# Autodesk Inventor assembly: IntakeRollerBar
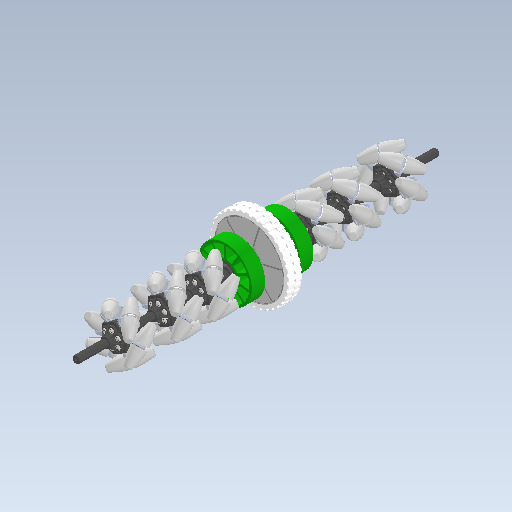
[picture p0: Inventor's stored thumbnail of the model, 512x512]
Saved by Autodesk Inventor 2020 (Build 240168000, 168)
## iProperties
Created: 2020-01-19
Part Number: IntakeRollerBar
Document SubType Name: Assembly
Designer: srini
Author: srini
## Documents named in this file (6)
- C:\Users\srini\Documents\FRC\2020\IntakeRollerBar.iam
- C:\Users\srini\Documents\FRC\2020\ThunderHex_27in.ipt
- C:\Users\srini\Documents\FRC\2020\MecWheels\4_Mecanum_Wheel_Left_217-3644.iam
- C:\Users\srini\Documents\FRC\2020\MecWheels\4_Mecanum_Wheel_Right_217-3645.iam
- C:\Users\srini\Documents\FRC\2020\am-3480 4IN 500Hex Compliant Wheel REV2.iam
- C:\Users\srini\Documents\FRC\2020\am-0940a 6 HiGrip wheel REV2_HexBore.iam
## Components (10 placed, 5 different names)
1. ThunderHex_27in:1 — Insert:1, Mate:1, Mate:3, Mate:5, Mate:7, Mate:9, Mate:11, Mate:13, Mate:15
2. 4_Mecanum_Wheel_Left_217-3644:1 [sub-assembly] — Mate:9, Mate:10
3. 4_Mecanum_Wheel_Left_217-3644:2 [sub-assembly] — Mate:7, Mate:8, Mate:10
4. 4_Mecanum_Wheel_Left_217-3644:3 [sub-assembly] — Mate:5, Mate:6, Mate:8
5. 4_Mecanum_Wheel_Right_217-3645:1 [sub-assembly] — Mate:13, Mate:14, Mate:16
6. 4_Mecanum_Wheel_Right_217-3645:2 [sub-assembly] — Mate:15, Mate:16
7. 4_Mecanum_Wheel_Right_217-3645:3 [sub-assembly] — Mate:11, Mate:12, Mate:14
8. am-3480 4IN 500Hex Compliant Wheel REV2:1 [sub-assembly] — Mate:3, Mate:4, Mate:12
9. am-3480 4IN 500Hex Compliant Wheel REV2:2 [sub-assembly] — Mate:1, Mate:2, Mate:6
10. am-0940a 6 HiGrip wheel REV2_HexBore:1 [sub-assembly] — Insert:1, Mate:2, Mate:4
## Relationships (17: Mate 16, Insert 1)
- Insert:1 (-342.9 mm): ThunderHex_27in:1 ↔ am-0940a 6 HiGrip wheel REV2_HexBore:1
- Mate:1: ThunderHex_27in:1 ↔ am-3480 4IN 500Hex Compliant Wheel REV2:2
- Mate:2 (12.7 mm): am-3480 4IN 500Hex Compliant Wheel REV2:2 ↔ am-0940a 6 HiGrip wheel REV2_HexBore:1
- Mate:3: ThunderHex_27in:1 ↔ am-3480 4IN 500Hex Compliant Wheel REV2:1
- Mate:4 (12.7 mm): am-3480 4IN 500Hex Compliant Wheel REV2:1 ↔ am-0940a 6 HiGrip wheel REV2_HexBore:1
- Mate:5: ThunderHex_27in:1 ↔ 4_Mecanum_Wheel_Left_217-3644:3
- Mate:6 (12.7 mm): 4_Mecanum_Wheel_Left_217-3644:3 ↔ am-3480 4IN 500Hex Compliant Wheel REV2:2
- Mate:7: ThunderHex_27in:1 ↔ 4_Mecanum_Wheel_Left_217-3644:2
- Mate:8 (12.7 mm): 4_Mecanum_Wheel_Left_217-3644:2 ↔ 4_Mecanum_Wheel_Left_217-3644:3
- Mate:9: ThunderHex_27in:1 ↔ 4_Mecanum_Wheel_Left_217-3644:1
- Mate:10 (31.75 mm): 4_Mecanum_Wheel_Left_217-3644:1 ↔ 4_Mecanum_Wheel_Left_217-3644:2
- Mate:11: ThunderHex_27in:1 ↔ 4_Mecanum_Wheel_Right_217-3645:3
- Mate:12 (12.7 mm): 4_Mecanum_Wheel_Right_217-3645:3 ↔ am-3480 4IN 500Hex Compliant Wheel REV2:1
- Mate:13: ThunderHex_27in:1 ↔ 4_Mecanum_Wheel_Right_217-3645:1
- Mate:14 (12.7 mm): 4_Mecanum_Wheel_Right_217-3645:1 ↔ 4_Mecanum_Wheel_Right_217-3645:3
- Mate:15: ThunderHex_27in:1 ↔ 4_Mecanum_Wheel_Right_217-3645:2
- Mate:16 (31.75 mm): 4_Mecanum_Wheel_Right_217-3645:1 ↔ 4_Mecanum_Wheel_Right_217-3645:2
